# Autodesk Inventor assembly: Top_Lever Assy
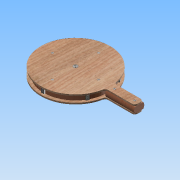
[picture p0: Inventor's stored thumbnail of the model, 180x180]
Saved by Autodesk Inventor 2018.1 (Build 221171000, 171)
## iProperties
Created: 2019-03-23
Part Number: Top_Lever Assy
Document SubType Name: Assembly
Designer: James
Author: James
## Documents named in this file (12)
- C:\Users\admin\Desktop\Ball-Machine\Top Level\Top_Lever Assy.iam
- C:\Users\admin\Desktop\Ball-Machine\Top Level\Top_Lever Centre.ipt
- C:\Users\admin\Desktop\Ball-Machine\Top Level\Top_Lever Side.ipt
- C:\Users\admin\Desktop\Ball-Machine\Top Level\Top_Lever Handle.ipt
- C:\Users\admin\Desktop\Ball-Machine\Top Level\Top_Lever Cable Tie.ipt
- C:\Users\admin\Desktop\Ball-Machine\Top Level\Din97 - 4x12 - Steel Wood Screw.ipt
- C:\Users\admin\Desktop\Ball-Machine\Top Level\PRB-256 - Standard Double Sealed Ball Bearing.ipt
- C:\Users\admin\Desktop\Ball-Machine\Top Level\Top_Lever Shaft.ipt
- C:\Users\admin\Desktop\Ball-Machine\Top Level\Top_Lever 2mm Spacer.ipt
- C:\Users\admin\Desktop\Ball-Machine\Top Level\Top_Lever End Piece.ipt
- C:\Users\admin\Desktop\Ball-Machine\Top Level\Socket Cap Screw - Standard - (A2) - M8 x 30.ipt
- C:\Users\admin\Desktop\Ball-Machine\Top Level\Socket Csk Screw - (A2) - M4 x  12.ipt
## Components (35 placed, 11 different names)
1. Top_Lever Centre:1 — Mate:1, Mate:2, Mate:3, Mate:4, Mate:5, Mate:6, Tangent:1, Mate:11, Mate:21, Flush:13
2. Top_Lever Side:1 — Flush:1, Flush:2, Flush:3, Mate:1, Mate:2, Mate:3, Flush:4, Mate:7, Flush:5, Mate:9, Mate:10, Flush:9, Mate:15, Mate:16, Flush:11, Mate:18, Mate:28
3. Top_Lever Side:2 — Mate:4, Flush:4, Mate:5, Mate:6, Mate:8, Angle:1, Flush:10, Mate:13, Mate:14, Flush:12, Mate:17, Mate:19, Mate:20
4. Top_Lever Handle:1 — Mate:7, Mate:8, Flush:5, Mate:9, Mate:10
5. Din97 - 4x12 - Steel Wood Screw:2 — Flush:8, Mate:14
6. Din97 - 4x12 - Steel Wood Screw:3 — Flush:8, Flush:10, Mate:13
7. Din97 - 4x12 - Steel Wood Screw:4 — Flush:7, Flush:9, Mate:15
8. Din97 - 4x12 - Steel Wood Screw:5 — Flush:7, Mate:16
9. PRB-256 - Standard Double Sealed Ball Bearing:1 — Mate:19, Mate:20, Mate:22, Mate:24
10. PRB-256 - Standard Double Sealed Ball Bearing:2 — Mate:25, Mate:26, Flush:13
11. Top_Lever Shaft:1 — Mate:21, Mate:22, Mate:23, Mate:26, Mate:27, Mate:29, Mate:30
12. Top_Lever 2mm Spacer:1 — Mate:23, Mate:24, Mate:25
13. Top_Lever End Piece:1 — Mate:27, Mate:28, Mate:31, Tangent:2
14. Socket Cap Screw - Standard - (A2) - M8 x 30:1 — Mate:29, Mate:30
15. Socket Csk Screw - (A2) - M4 x  12:1 — Mate:31, Tangent:2
16. Din97 - 4x12 - Steel Wood Screw:1 — Mate:12, Flush:6
17. Top_Lever Cable Tie:1 — Tangent:1, Mate:11, Angle:1, Mate:12, Flush:6
18. Din97 - 4x12 - Steel Wood Screw:6
19. Top_Lever Cable Tie:2
20. Din97 - 4x12 - Steel Wood Screw:7
21. Top_Lever Cable Tie:3
22. Din97 - 4x12 - Steel Wood Screw:8
23. Top_Lever Cable Tie:4
24. Din97 - 4x12 - Steel Wood Screw:9
25. Top_Lever Cable Tie:5
26. Din97 - 4x12 - Steel Wood Screw:10
27. Top_Lever Cable Tie:6
28. Din97 - 4x12 - Steel Wood Screw:11 — Flush:11, Mate:18
29. Din97 - 4x12 - Steel Wood Screw:12 — Flush:12, Mate:17
30. Din97 - 4x12 - Steel Wood Screw:13
31. Din97 - 4x12 - Steel Wood Screw:14
32. Din97 - 4x12 - Steel Wood Screw:15
33. Din97 - 4x12 - Steel Wood Screw:16
34. Din97 - 4x12 - Steel Wood Screw:17
35. Din97 - 4x12 - Steel Wood Screw:18
## Component patterns: (6 elements, first: Din97 - 4x12 - Steel Wood Screw:1 + Top_Lever Cable Tie:1), (4 elements, first: Din97 - 4x12 - Steel Wood Screw:11 + Din97 - 4x12 - Steel Wood Screw:12)
## Relationships (47: Mate 31, Flush 13, Tangent 2, Angle 1)
- Flush:1: Top_Lever Side:1
- Flush:2: Top_Lever Side:1
- Flush:3: Top_Lever Side:1
- Mate:1: Top_Lever Centre:1 ↔ Top_Lever Side:1
- Mate:2: Top_Lever Centre:1 ↔ Top_Lever Side:1
- Mate:3: Top_Lever Centre:1 ↔ Top_Lever Side:1
- Mate:4: Top_Lever Centre:1 ↔ Top_Lever Side:2
- Flush:4: Top_Lever Side:1 ↔ Top_Lever Side:2
- Mate:5: Top_Lever Centre:1 ↔ Top_Lever Side:2
- Mate:6: Top_Lever Centre:1 ↔ Top_Lever Side:2
- Mate:7: Top_Lever Side:1 ↔ Top_Lever Handle:1
- Mate:8: Top_Lever Side:2 ↔ Top_Lever Handle:1
- Flush:5: Top_Lever Side:1 ↔ Top_Lever Handle:1
- Mate:9: Top_Lever Side:1 ↔ Top_Lever Handle:1
- Mate:10: Top_Lever Side:1 ↔ Top_Lever Handle:1
- Tangent:1: Top_Lever Centre:1 ↔ Top_Lever Cable Tie:1
- Mate:11: Top_Lever Centre:1 ↔ Top_Lever Cable Tie:1
- Angle:1 (0 deg): Top_Lever Side:2 ↔ Top_Lever Cable Tie:1
- Mate:12: Din97 - 4x12 - Steel Wood Screw:1 ↔ Top_Lever Cable Tie:1
- Flush:6: Din97 - 4x12 - Steel Wood Screw:1 ↔ Top_Lever Cable Tie:1
- Flush:7: Din97 - 4x12 - Steel Wood Screw:4 ↔ Din97 - 4x12 - Steel Wood Screw:5
- Flush:8: Din97 - 4x12 - Steel Wood Screw:2 ↔ Din97 - 4x12 - Steel Wood Screw:3
- Flush:9: Top_Lever Side:1 ↔ Din97 - 4x12 - Steel Wood Screw:4
- Flush:10: Top_Lever Side:2 ↔ Din97 - 4x12 - Steel Wood Screw:3
- Mate:13: Top_Lever Side:2 ↔ Din97 - 4x12 - Steel Wood Screw:3
- Mate:14: Top_Lever Side:2 ↔ Din97 - 4x12 - Steel Wood Screw:2
- Mate:15: Top_Lever Side:1 ↔ Din97 - 4x12 - Steel Wood Screw:4
- Mate:16: Top_Lever Side:1 ↔ Din97 - 4x12 - Steel Wood Screw:5
- Flush:11: Top_Lever Side:1 ↔ Din97 - 4x12 - Steel Wood Screw:11
- Flush:12: Top_Lever Side:2 ↔ Din97 - 4x12 - Steel Wood Screw:12
- Mate:17: Top_Lever Side:2 ↔ Din97 - 4x12 - Steel Wood Screw:12
- Mate:18: Top_Lever Side:1 ↔ Din97 - 4x12 - Steel Wood Screw:11
- Mate:19: Top_Lever Side:2 ↔ PRB-256 - Standard Double Sealed Ball Bearing:1
- Mate:20: Top_Lever Side:2 ↔ PRB-256 - Standard Double Sealed Ball Bearing:1
- Mate:21: Top_Lever Centre:1 ↔ Top_Lever Shaft:1
- Mate:22: PRB-256 - Standard Double Sealed Ball Bearing:1 ↔ Top_Lever Shaft:1
- Mate:23: Top_Lever Shaft:1 ↔ Top_Lever 2mm Spacer:1
- Mate:24: PRB-256 - Standard Double Sealed Ball Bearing:1 ↔ Top_Lever 2mm Spacer:1
- Mate:25: PRB-256 - Standard Double Sealed Ball Bearing:2 ↔ Top_Lever 2mm Spacer:1
- Mate:26: PRB-256 - Standard Double Sealed Ball Bearing:2 ↔ Top_Lever Shaft:1
- Flush:13: Top_Lever Centre:1 ↔ PRB-256 - Standard Double Sealed Ball Bearing:2
- Mate:27: Top_Lever Shaft:1 ↔ Top_Lever End Piece:1
- Mate:28: Top_Lever Side:1 ↔ Top_Lever End Piece:1
- Mate:29: Top_Lever Shaft:1 ↔ Socket Cap Screw - Standard - (A2) - M8 x 30:1
- Mate:30 (15 mm): Top_Lever Shaft:1 ↔ Socket Cap Screw - Standard - (A2) - M8 x 30:1
- Mate:31: Top_Lever End Piece:1 ↔ Socket Csk Screw - (A2) - M4 x  12:1
- Tangent:2: Top_Lever End Piece:1 ↔ Socket Csk Screw - (A2) - M4 x  12:1
